# Autodesk Inventor assembly: box_full
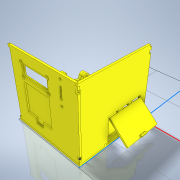
[picture p0: Inventor's stored thumbnail of the model, 180x180]
Saved by Autodesk Inventor 2020 (Build 240168000, 168)
## iProperties
Created: 2020-02-25
Part Number: box_full
Document SubType Name: Assembly
Designer: Luka
Author: Luka
## Documents named in this file (9)
- C:\Users\Luka\Desktop\box_full.iam
- C:\Users\Luka\Desktop\box_bottom.ipt
- C:\Users\Luka\Desktop\box_right.ipt
- C:\Users\Luka\Desktop\box_front.ipt
- C:\Users\Luka\Desktop\coin_slot.ipt
- C:\Users\Luka\Desktop\box_door.ipt
- C:\Users\Luka\Desktop\box_full\Design Accelerator\Bolted Connection2.iam
- C:\Users\Luka\Desktop\box_full\Design Accelerator\Bolted Connection3.iam
- C:\Users\Luka\Desktop\box_full\Design Accelerator\Bolted Connection4.iam
## Components (8 placed, 6 different names)
1. box_bottom:2 — Rigid:2, Mate:1, Mate:2, Mate:3, Mate:4, Mate:5, Mate:6
2. box_front:1 — Rigid:3, Rotational:2
3. box_right:1 — Rigid:2, Rigid:3, Rotational:3
4. coin_slot:1 — Rotational:2
5. box_door:1 — Rotational:3
6. Bolted Connection:1 [sub-assembly] — Mate:1, Mate:2
7. Bolted Connection:2 [sub-assembly] — Mate:3, Mate:4
8. Bolted Connection:3 [sub-assembly] — Mate:5, Mate:6
## Relationships (10: Mate 6, WeldJoint 2, RevoluteJoint 2)
- Rigid:2 [WeldJoint]: box_bottom:2 ↔ box_right:1
- Rigid:3 [WeldJoint]: box_front:1 ↔ box_right:1
- Rotational:2 [RevoluteJoint]: box_front:1 ↔ coin_slot:1
- Rotational:3 [RevoluteJoint]: box_right:1 ↔ box_door:1
- Mate:1: box_bottom:2 ↔ Bolted Connection:1
- Mate:2: box_bottom:2 ↔ Bolted Connection:1
- Mate:3: box_bottom:2 ↔ Bolted Connection:2
- Mate:4: box_bottom:2 ↔ Bolted Connection:2
- Mate:5: box_bottom:2 ↔ Bolted Connection:3
- Mate:6: box_bottom:2 ↔ Bolted Connection:3
